# Autodesk Inventor assembly: femur +horn
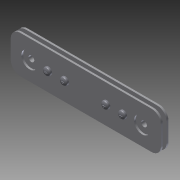
[picture p0: Inventor's stored thumbnail of the model, 180x180]
Saved by Autodesk Inventor 2012 (Build 160160000, 160)
## iProperties
Created: 2013-12-07
Part Number: femur +horn
Document SubType Name: Assembly
Designer: Irwan Haryanto
Author: Irwan Haryanto
## Documents named in this file (5)
- D:\Revenant\robot baru 2014\femur +horn.iam
- D:\Revenant\robot baru 2014\femur 6 cm.ipt
- D:\Revenant\robot baru 2014\Horn.ipt
- D:\Revenant\robot baru 2014\femur +horn\Design Accelerator\Bolted Connection1.iam
- D:\Revenant\robot baru 2014\femur +horn\Design Accelerator\Bolted Connection2.iam
## Components (6 placed, 3 different names)
1. femur 6 cm:1 — Insert:5, Insert:6, Insert:7, Insert:8
2. femur 6 cm:2 — Insert:1, Insert:2, Insert:3, Insert:4, Mate:1, Mate:3
3. Horn:1 — Insert:3, Insert:4, Insert:7, Insert:8, Mate:2
4. Horn:2 — Insert:1, Insert:2, Insert:5, Insert:6, Mate:4
5. Bolted Connection:1 [sub-assembly] — Mate:1, Mate:2
6. Bolted Connection:2 [sub-assembly] — Mate:3, Mate:4
## Relationships (12: Insert 8, Mate 4)
- Insert:1: femur 6 cm:2 ↔ Horn:2
- Insert:2: femur 6 cm:2 ↔ Horn:2
- Insert:3: femur 6 cm:2 ↔ Horn:1
- Insert:4: femur 6 cm:2 ↔ Horn:1
- Insert:5: femur 6 cm:1 ↔ Horn:2
- Insert:6: femur 6 cm:1 ↔ Horn:2
- Insert:7: femur 6 cm:1 ↔ Horn:1
- Insert:8: femur 6 cm:1 ↔ Horn:1
- Mate:1: femur 6 cm:2 ↔ Bolted Connection:1
- Mate:2: Horn:1 ↔ Bolted Connection:1
- Mate:3: femur 6 cm:2 ↔ Bolted Connection:2
- Mate:4: Horn:2 ↔ Bolted Connection:2
